# Autodesk Inventor assembly: Разъём с предохранителем и выключателем
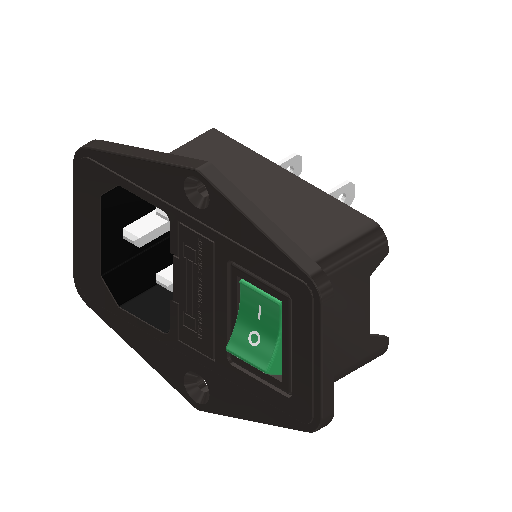
[picture p0: Inventor's stored thumbnail of the model, 512x512]
Saved by Autodesk Inventor 2022 (Build 260153000, 153)
## iProperties
Created: 2021-05-30
Part Number: Разъём с предохранителем и выключателем
Document SubType Name: Assembly
Designer: Mikhail
Author: Mikhail
## Documents named in this file (3)
- D:\YandexDisk\РЕЗЕРВ\Делета робот\3Д модели\Разъём с выключателем и предохранителем\Разъём с предохранителем и выключателем.iam
- D:\YandexDisk\РЕЗЕРВ\Делета робот\3Д модели\Разъём с выключателем и предохранителем\ARCOLECTRIC_H8600VB.ipt
- D:\YandexDisk\РЕЗЕРВ\Делета робот\3Д модели\Разъём с выключателем и предохранителем\Разъём.ipt
## Components (2 placed, 2 different names)
1. ARCOLECTRIC_H8600VB:1 — Заподлицо:1, Заподлицо:2, Заподлицо:3
2. Разъём:1 — Заподлицо:1, Заподлицо:2, Заподлицо:3
## Relationships (3: Flush 3)
- Заподлицо:1 [Flush]: ARCOLECTRIC_H8600VB:1 ↔ Разъём:1
- Заподлицо:2 [Flush] (5 mm): ARCOLECTRIC_H8600VB:1 ↔ Разъём:1
- Заподлицо:3 [Flush] (3.8 mm): ARCOLECTRIC_H8600VB:1 ↔ Разъём:1
